# Autodesk Inventor assembly: 4_Bar_Linkage
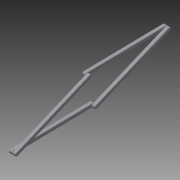
[picture p0: Inventor's stored thumbnail of the model, 180x180]
Saved by Autodesk Inventor 2015 (Build 190159000, 159)
## iProperties
Created: 2015-04-08
Part Number: 4_Bar_Linkage
Document SubType Name: Assembly
Designer: WASHHSST
Author: WASHHSST
## Documents named in this file (3)
- C:\Users\washhsst\Documents\GitHub\myWork\4_Bar_Linkage.iam
- C:\Users\washhsst\Documents\GitHub\myWork\4_Bar_Linkage\bar.ipt
- C:\Users\washhsst\Documents\GitHub\myWork\4_Bar_Linkage\pin.ipt
## Components (8 placed, 2 different names)
1. bar:1 — Insert:5, Insert:9, Mate:1
2. pin:1 — Insert:4, Insert:5
3. bar:2 — Insert:3, Insert:4, Mate:2
4. pin:2 — Insert:2, Insert:7
5. bar:3 — Insert:1, Insert:2, Mate:1
6. pin:3 — Insert:1, Insert:3
7. bar:4 — Insert:7, Insert:8, Mate:2
8. pin:4 — Insert:8, Insert:9
## Relationships (10: Insert 8, Mate 2)
- Insert:1: bar:3 ↔ pin:3
- Insert:2: pin:2 ↔ bar:3
- Insert:3: bar:2 ↔ pin:3
- Insert:4: pin:1 ↔ bar:2
- Insert:5: bar:1 ↔ pin:1
- Insert:7: pin:2 ↔ bar:4
- Insert:8: bar:4 ↔ pin:4
- Insert:9: bar:1 ↔ pin:4
- Mate:1: bar:1 ↔ bar:3
- Mate:2: bar:2 ↔ bar:4
